# Autodesk Inventor assembly: SYS-ASM-0000-Main
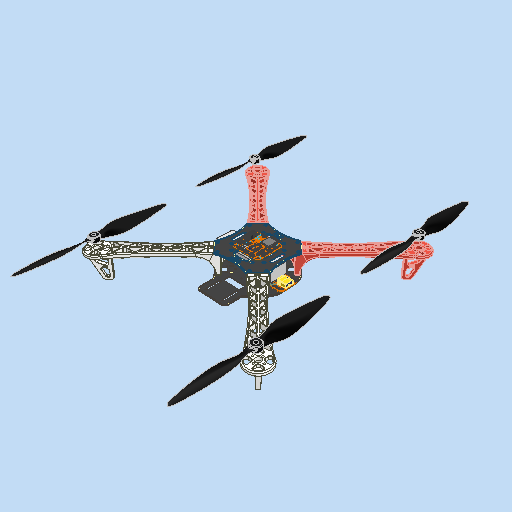
[picture p0: Inventor's stored thumbnail of the model, 512x512]
Saved by Autodesk Inventor 2026 (Build 300175000, 175)
## iProperties
Created: 2026-07-22
Part Number: SYS-ASM-0000-Main
Document SubType Name: Assembly
Designer: Pacman Ng
Author: Pacman Ng
## Documents named in this file (6)
- D:\OneDrive_MSFT\Work\Drone_Research\3d_models\Full_body\SYS-ASM-0000-Main.iam
- D:\OneDrive_MSFT\Work\Drone_Research\3d_models\Full_body\MEC-ASM-1000-F450_Frame.iam
- D:\OneDrive_MSFT\Work\Drone_Research\3d_models\Full_body\PWR-PRT-2001-Lipo3S.ipt
- D:\OneDrive_MSFT\Work\Drone_Research\3d_models\Full_body\PCB-ASM-6000-Power_Monitor.iam
- D:\OneDrive_MSFT\Work\Drone_Research\3d_models\Full_body\AVI-PRT-5001-Propeller_10x45.ipt
- D:\OneDrive_MSFT\Work\Drone_Research\3d_models\Full_body\PCB-ASM-3000-FC_v02.iam
## Components (8 placed, 5 different names)
1. AVI-PRT-5001-Propeller_10x45:1
2. AVI-PRT-5001-Propeller_10x45:2
3. AVI-PRT-5001-Propeller_10x45:3
4. AVI-PRT-5001-Propeller_10x45:4
5. MEC-ASM-1000-F450_Frame:1 [sub-assembly] — Mate:1, Mate:2, Mate:3
6. PCB-ASM-6000-Power_Monitor:1 [sub-assembly] — Mate:1, Mate:2, Mate:3
7. PWR-PRT-2001-Lipo3S:1
8. PCB-ASM-3000-FC_v02:1 [sub-assembly]
## Relationships (3: Mate 3)
- Mate:1: MEC-ASM-1000-F450_Frame:1 ↔ PCB-ASM-6000-Power_Monitor:1
- Mate:2 (-0.8 mm): MEC-ASM-1000-F450_Frame:1 ↔ PCB-ASM-6000-Power_Monitor:1
- Mate:3 (-12.65 mm): MEC-ASM-1000-F450_Frame:1 ↔ PCB-ASM-6000-Power_Monitor:1
